# Autodesk Inventor assembly: LeftFootUnit
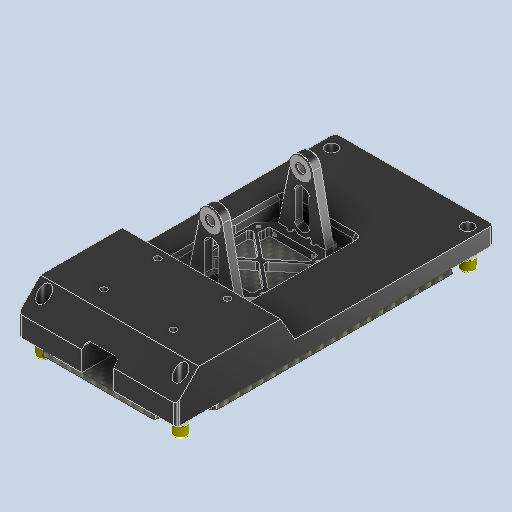
[picture p0: Inventor's stored thumbnail of the model, 512x512]
Saved by Autodesk Inventor 2024.2 (Build 282272000, 272)
## iProperties
Created: 2024-01-07
Part Number: LeftFootUnit
Document SubType Name: Assembly
Designer: Masato Kubotera
Mass: 227.586 g
Surface Area: 1232.19 cm^2
Volume: 155.4 cm^3
Density: 1.46452 g/cm^3
Author: Masato Kubotera
## Documents named in this file (14)
- C:\Users\masato\OneDrive - Chiba Institute of Technology\CIT Brains\RoboCup2024\Mechanic\SUSTAINA-OP2-DEV - 作業\NativeFiles\Boby\LowerLimb\Feet\LeftFootUnit.iam
- C:\Users\masato\OneDrive - Chiba Institute of Technology\CIT Brains\RoboCup2024\Mechanic\SUSTAINA-OP2-DEV - 作業\NativeFiles\Boby\LowerLimb\LegRollSliderFrame.ipt
- C:\Users\masato\OneDrive - Chiba Institute of Technology\CIT Brains\RoboCup2024\Mechanic\SUSTAINA-OP2-DEV - 作業\NativeFiles\Boby\COTS\Bushes\GFM-0608-06.ipt
- C:\Users\masato\OneDrive - Chiba Institute of Technology\CIT Brains\RoboCup2024\Mechanic\SUSTAINA-OP2-DEV - 作業\NativeFiles\Boby\COTS\Washers\Metal\UUW-0614-05H.ipt
- C:\Users\masato\OneDrive - Chiba Institute of Technology\CIT Brains\RoboCup2024\Mechanic\SUSTAINA-OP2-DEV - 作業\NativeFiles\Boby\COTS\Screws\CapScrew\UC-0310.ipt
- C:\Users\masato\OneDrive - Chiba Institute of Technology\CIT Brains\RoboCup2024\Mechanic\SUSTAINA-OP2-DEV - 作業\NativeFiles\Boby\LowerLimb\Feet\FootBraceFrame.ipt
- C:\Users\masato\OneDrive - Chiba Institute of Technology\CIT Brains\RoboCup2024\Mechanic\SUSTAINA-OP2-DEV - 作業\NativeFiles\Boby\LowerLimb\Feet\FootSoleFrame.ipt
- C:\Users\masato\OneDrive - Chiba Institute of Technology\CIT Brains\RoboCup2024\Mechanic\SUSTAINA-OP2-DEV - 作業\NativeFiles\Boby\COTS\Screws\CapScrew\UC-0308.ipt
- C:\Users\masato\OneDrive - Chiba Institute of Technology\CIT Brains\RoboCup2024\Mechanic\SUSTAINA-OP2-DEV - 作業\NativeFiles\Boby\COTS\MisumiComponents\URLM8\URLM8.iam
- C:\Users\masato\OneDrive - Chiba Institute of Technology\CIT Brains\RoboCup2024\Mechanic\SUSTAINA-OP2-DEV - 作業\NativeFiles\Boby\COTS\ElectronicComponents\SC700-40kg.ipt
- C:\Users\masato\OneDrive - Chiba Institute of Technology\CIT Brains\RoboCup2024\Mechanic\SUSTAINA-OP2-DEV - 作業\NativeFiles\Boby\COTS\Screws\CapScrew\UC-0306.ipt
- C:\Users\masato\OneDrive - Chiba Institute of Technology\CIT Brains\RoboCup2024\Mechanic\SUSTAINA-OP2-DEV - 作業\NativeFiles\Boby\CustomPCBs\Quad-Load-Cell-Amplifier-to-RS-485-Conv-Module.ipt
- C:\Users\masato\OneDrive - Chiba Institute of Technology\CIT Brains\RoboCup2024\Mechanic\SUSTAINA-OP2-DEV - 作業\NativeFiles\Boby\LowerLimb\Feet\LeftFootCover.ipt
- C:\Users\masato\OneDrive - Chiba Institute of Technology\CIT Brains\RoboCup2024\Mechanic\SUSTAINA-OP2-DEV - 作業\NativeFiles\Boby\COTS\Washers\Resin\TT-0614-05.ipt
## Components (40 placed, 13 different names)
1. LegRollSliderFrame:1 — Mate:1, Angle:1, Flush:2, Flush:3, Insert:1, Insert:3, Insert:7, Insert:8, Insert:11, Insert:12, Mate:2
2. LegRollSliderFrame:2 — Flush:2, Flush:3, Insert:2, Insert:4, Insert:9, Insert:10, Insert:13, Insert:14
3. FootBraceFrame:1 — Insert:11, Insert:12, Insert:13, Insert:14, Insert:15, Insert:16, Insert:17, Insert:18
4. FootSoleFrame:1 — Insert:15, Insert:16, Insert:17, Insert:18, Insert:19, Insert:20, Insert:21, Insert:22, Insert:23, Insert:24, Insert:25, Insert:26, Insert:27, Insert:28, Insert:29, Insert:30, Flush:4, Flush:5, Flush:6, Insert:41, Insert:42, Insert:43, Insert:44, Insert:45, Insert:46, Insert:47, Insert:48
5. Quad-Load-Cell-Amplifier-to-RS-485-Conv-Module:1 — Insert:39, Insert:40
6. LeftFootCover:1 — Insert:39, Insert:40, Flush:4, Flush:5, Flush:6
7. GFM-0608-06:1 — Insert:1
8. GFM-0608-06:2 — Insert:2
9. SC700-40kg:1 — Insert:23, Insert:24, Insert:31, Insert:35
10. SC700-40kg:2 — Insert:25, Insert:26, Insert:32, Insert:36
11. SC700-40kg:3 — Insert:27, Insert:28, Insert:33, Insert:37
12. SC700-40kg:4 — Insert:29, Insert:30, Insert:34, Insert:38
13. UC-0306:1 — Insert:35
14. UC-0306:2 — Insert:36
15. UC-0306:3 — Insert:37
16. UC-0306:4 — Insert:38
17. UC-0310:5 — Insert:41
18. UC-0310:6 — Insert:42
19. UC-0310:7 — Insert:43
20. UC-0310:8 — Insert:44
21. UC-0308:5 — Insert:45
22. UC-0308:6 — Insert:46
23. UC-0308:7 — Insert:47
24. UC-0308:8 — Insert:48
25. UC-0310:1 — Insert:7
26. UC-0310:2 — Insert:8
27. UC-0310:3 — Insert:9
28. UC-0310:4 — Insert:10
29. UC-0308:1 — Insert:19
30. UC-0308:2 — Insert:20
31. UC-0308:3 — Insert:21
32. UC-0308:4 — Insert:22
33. URLM8:1 [sub-assembly] — Insert:31
34. URLM8:2 [sub-assembly] — Insert:32
35. URLM8:3 [sub-assembly] — Insert:33
36. URLM8:4 [sub-assembly] — Insert:34
37. TT-0614-05:2 — Insert:3, Insert:5
38. TT-0614-05:1 — Insert:4, Insert:6
39. UUW-0614-05H:1 — Insert:5
40. UUW-0614-05H:2 — Insert:6
## Relationships (56: Insert 48, Flush 5, Mate 2, Angle 1)
- Mate:1: LegRollSliderFrame:1
- Angle:1 (180 deg): LegRollSliderFrame:1
- Flush:2: LegRollSliderFrame:1 ↔ LegRollSliderFrame:2
- Flush:3: LegRollSliderFrame:1 ↔ LegRollSliderFrame:2
- Insert:1: LegRollSliderFrame:1 ↔ GFM-0608-06:1
- Insert:2: LegRollSliderFrame:2 ↔ GFM-0608-06:2
- Insert:3: LegRollSliderFrame:1 ↔ TT-0614-05:2
- Insert:4: LegRollSliderFrame:2 ↔ TT-0614-05:1
- Insert:5: TT-0614-05:2 ↔ UUW-0614-05H:1
- Insert:6: TT-0614-05:1 ↔ UUW-0614-05H:2
- Insert:7: LegRollSliderFrame:1 ↔ UC-0310:1
- Insert:8: LegRollSliderFrame:1 ↔ UC-0310:2
- Insert:9: LegRollSliderFrame:2 ↔ UC-0310:3
- Insert:10: LegRollSliderFrame:2 ↔ UC-0310:4
- Insert:11: LegRollSliderFrame:1 ↔ FootBraceFrame:1
- Insert:12: LegRollSliderFrame:1 ↔ FootBraceFrame:1
- Insert:13: LegRollSliderFrame:2 ↔ FootBraceFrame:1
- Insert:14: LegRollSliderFrame:2 ↔ FootBraceFrame:1
- Mate:2 (16 mm): LegRollSliderFrame:1
- Insert:15: FootBraceFrame:1 ↔ FootSoleFrame:1
- Insert:16: FootBraceFrame:1 ↔ FootSoleFrame:1
- Insert:17: FootBraceFrame:1 ↔ FootSoleFrame:1
- Insert:18: FootBraceFrame:1 ↔ FootSoleFrame:1
- Insert:19: FootSoleFrame:1 ↔ UC-0308:1
- Insert:20: FootSoleFrame:1 ↔ UC-0308:2
- Insert:21: FootSoleFrame:1 ↔ UC-0308:3
- Insert:22: FootSoleFrame:1 ↔ UC-0308:4
- Insert:23: FootSoleFrame:1 ↔ SC700-40kg:1
- Insert:24: FootSoleFrame:1 ↔ SC700-40kg:1
- Insert:25: FootSoleFrame:1 ↔ SC700-40kg:2
- Insert:26: FootSoleFrame:1 ↔ SC700-40kg:2
- Insert:27: FootSoleFrame:1 ↔ SC700-40kg:3
- Insert:28: FootSoleFrame:1 ↔ SC700-40kg:3
- Insert:29: FootSoleFrame:1 ↔ SC700-40kg:4
- Insert:30: FootSoleFrame:1 ↔ SC700-40kg:4
- Insert:31: SC700-40kg:1 ↔ URLM8:1
- Insert:32: SC700-40kg:2 ↔ URLM8:2
- Insert:33: SC700-40kg:3 ↔ URLM8:3
- Insert:34: SC700-40kg:4 ↔ URLM8:4
- Insert:35: SC700-40kg:1 ↔ UC-0306:1
- Insert:36: SC700-40kg:2 ↔ UC-0306:2
- Insert:37: SC700-40kg:3 ↔ UC-0306:3
- Insert:38: SC700-40kg:4 ↔ UC-0306:4
- Insert:39: Quad-Load-Cell-Amplifier-to-RS-485-Conv-Module:1 ↔ LeftFootCover:1
- Insert:40: Quad-Load-Cell-Amplifier-to-RS-485-Conv-Module:1 ↔ LeftFootCover:1
- Flush:4: FootSoleFrame:1 ↔ LeftFootCover:1
- Flush:5: FootSoleFrame:1 ↔ LeftFootCover:1
- Flush:6: FootSoleFrame:1 ↔ LeftFootCover:1
- Insert:41: FootSoleFrame:1 ↔ UC-0310:5
- Insert:42: FootSoleFrame:1 ↔ UC-0310:6
- Insert:43: FootSoleFrame:1 ↔ UC-0310:7
- Insert:44: FootSoleFrame:1 ↔ UC-0310:8
- Insert:45: FootSoleFrame:1 ↔ UC-0308:5
- Insert:46: FootSoleFrame:1 ↔ UC-0308:6
- Insert:47: FootSoleFrame:1 ↔ UC-0308:7
- Insert:48: FootSoleFrame:1 ↔ UC-0308:8
